# Autodesk Inventor assembly: rotor_core
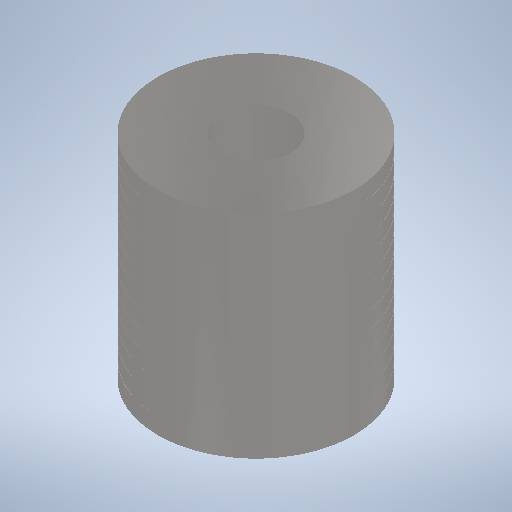
[picture p0: Inventor's stored thumbnail of the model, 512x512]
Saved by Autodesk Inventor 2025 (Build 290162000, 162)
## iProperties
Created: 2026-08-03
Part Number: rotor_core
Document SubType Name: Assembly
Designer: zzapa
Author: zzapa
## Documents named in this file (2)
- C:\Users\zzapa\Desktop\Projekty\elektronika\engine-project\model\assemblies\rotor_core.iam
- C:\Users\zzapa\Documents\Inventor\Content Center Files\R2025\pl-PL\DIN 9021\DIN 9021 - 10,5.ipt
## Components (13 placed, 1 different names)
1. DIN 9021 10,5:1 — Zestawiające:1, Zestawiające:2
2. DIN 9021 10,5:2
3. DIN 9021 10,5:3
4. DIN 9021 10,5:4
5. DIN 9021 10,5:5
6. DIN 9021 10,5:6
7. DIN 9021 10,5:7
8. DIN 9021 10,5:8
9. DIN 9021 10,5:9
10. DIN 9021 10,5:10
11. DIN 9021 10,5:11
12. DIN 9021 10,5:12
13. DIN 9021 10,5:13
## Component patterns: (13 elements, first: DIN 9021 10,5:1)
## Relationships (2: Mate 2)
- Zestawiające:1 [Mate]: DIN 9021 10,5:1
- Zestawiające:2 [Mate]: DIN 9021 10,5:1
